# Autodesk Inventor assembly: パネル型スカラアーム
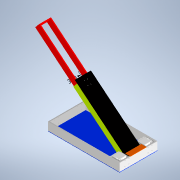
[picture p0: Inventor's stored thumbnail of the model, 180x180]
Saved by Autodesk Inventor 2022 (Build 260153000, 153)
## iProperties
Created: 2022-10-17
Part Number: パネル型スカラアーム
Document SubType Name: Assembly
Designer: tdn82
Mass: 1402.96 g
Surface Area: 5352.73 cm^2
Volume: 859.492 cm^3
Density: 1.63232 g/cm^3
Author: tdn82
## Documents named in this file (14)
- C:\Users\tdn82\OneDrive\ドキュメント\Inventor\卒業研究パネル型スカラアーム\GrabCAD\panel-type-scalar-arm\パネル型スカラアーム\パネル型スカラアーム.iam
- C:\Users\tdn82\OneDrive\ドキュメント\Inventor\卒業研究パネル型スカラアーム\GrabCAD\panel-type-scalar-arm\パネル型スカラアーム\縦長フラットバー.ipt
- C:\Users\tdn82\OneDrive\ドキュメント\Inventor\卒業研究パネル型スカラアーム\GrabCAD\panel-type-scalar-arm\パネル型スカラアーム\横長フラットバー.ipt
- C:\Users\tdn82\OneDrive\ドキュメント\Inventor\卒業研究パネル型スカラアーム\GrabCAD\panel-type-scalar-arm\パネル型スカラアーム\サーボモータB3M-SC-1170-AB3M1100_scale.ipt
- C:\Users\tdn82\OneDrive\ドキュメント\Inventor\卒業研究パネル型スカラアーム\GrabCAD\panel-type-scalar-arm\パネル型スカラアーム\後ろカバー.ipt
- C:\Users\tdn82\OneDrive\ドキュメント\Inventor\卒業研究パネル型スカラアーム\GrabCAD\panel-type-scalar-arm\パネル型スカラアーム\横長3rdフラットバー.ipt
- C:\Users\tdn82\OneDrive\ドキュメント\Inventor\卒業研究パネル型スカラアーム\GrabCAD\panel-type-scalar-arm\パネル型スカラアーム\縦長3rdフラットバー.ipt
- C:\Users\tdn82\OneDrive\ドキュメント\Inventor\卒業研究パネル型スカラアーム\GrabCAD\panel-type-scalar-arm\パネル型スカラアーム\１段目アーム.iam
- C:\Users\tdn82\OneDrive\ドキュメント\Inventor\卒業研究パネル型スカラアーム\GrabCAD\panel-type-scalar-arm\パネル型スカラアーム\横長2ndフラットバー.ipt
- C:\Users\tdn82\OneDrive\ドキュメント\Inventor\卒業研究パネル型スカラアーム\GrabCAD\panel-type-scalar-arm\パネル型スカラアーム\横長3rdフラットバー上.ipt
- C:\Users\tdn82\OneDrive\ドキュメント\Inventor\卒業研究パネル型スカラアーム\GrabCAD\panel-type-scalar-arm\パネル型スカラアーム\サーボモータ固定２軸目.ipt
- C:\Users\tdn82\OneDrive\ドキュメント\Inventor\卒業研究パネル型スカラアーム\GrabCAD\panel-type-scalar-arm\パネル型スカラアーム\前上下カバー.ipt
- C:\Users\tdn82\OneDrive\ドキュメント\Inventor\卒業研究パネル型スカラアーム\GrabCAD\panel-type-scalar-arm\パネル型スカラアーム\前カバー中盤.ipt
- C:\Users\tdn82\OneDrive\ドキュメント\Inventor\卒業研究パネル型スカラアーム\GrabCAD\panel-type-scalar-arm\パネル型スカラアーム\黒棒.ipt
## Components (18 placed, 13 different names)
1. 縦長フラットバー:1 — メイト:1, フラッシュ:1, フラッシュ:2, フラッシュ:3, メイト:2, メイト:3, メイト:4, メイト:12
2. 縦長フラットバー:2 — メイト:5, メイト:6, メイト:7, メイト:8, 挿入:1, 挿入:2, 挿入:3, 挿入:4, メイト:22, メイト:24, メイト:29, メイト:31
3. 横長フラットバー:1 — メイト:2, メイト:3, メイト:4, メイト:5, メイト:6, メイト:11, メイト:23
4. 横長フラットバー:3 — メイト:7, メイト:8, メイト:25
5. サーボモータB3M-SC-1170-AB3M1100_scale:2 — 挿入:7, 挿入:8, 挿入:9
6. 後ろカバー:1 — メイト:11, メイト:12
7. 横長3rdフラットバー:2 — メイト:18, メイト:19, 挿入:7
8. 縦長3rdフラットバー:1 — メイト:18, メイト:19, メイト:20, メイト:21
9. １段目アーム:1 [sub-assembly] — 挿入:1, 挿入:2, 挿入:12
10. １段目アーム:2 [sub-assembly] — 挿入:3, 挿入:4, 挿入:13
11. 横長2ndフラットバー:1 — フラッシュ:4, 挿入:13
12. 横長2ndフラットバー:2 — フラッシュ:4, メイト:26, メイト:27, メイト:28, 挿入:12
13. 横長3rdフラットバー上:1 — メイト:20, メイト:21
14. 前上下カバー:1 — メイト:22, メイト:23, メイト:30
15. 前上下カバー:2 — メイト:24, メイト:25
16. 前カバー中盤:1 — メイト:26, メイト:27, メイト:28, 挿入:10, 挿入:11
17. サーボモータ固定２軸目:1 — 挿入:8, 挿入:9, 挿入:10, 挿入:11
18. 黒棒:1 — メイト:29, メイト:30, メイト:31
## Relationships (39: Mate 24, Insert 11, Flush 4)
- メイト:1 [Mate]: 縦長フラットバー:1
- フラッシュ:1 [Flush]: 縦長フラットバー:1
- フラッシュ:2 [Flush]: 縦長フラットバー:1
- フラッシュ:3 [Flush]: 縦長フラットバー:1
- メイト:2 [Mate]: 縦長フラットバー:1 ↔ 横長フラットバー:1
- メイト:3 [Mate]: 縦長フラットバー:1 ↔ 横長フラットバー:1
- メイト:4 [Mate]: 縦長フラットバー:1 ↔ 横長フラットバー:1
- メイト:5 [Mate]: 縦長フラットバー:2 ↔ 横長フラットバー:1
- メイト:6 [Mate]: 縦長フラットバー:2 ↔ 横長フラットバー:1
- メイト:7 [Mate]: 縦長フラットバー:2 ↔ 横長フラットバー:3
- メイト:8 [Mate]: 縦長フラットバー:2 ↔ 横長フラットバー:3
- メイト:11 [Mate]: 横長フラットバー:1 ↔ 後ろカバー:1
- メイト:12 [Mate]: 縦長フラットバー:1 ↔ 後ろカバー:1
- メイト:18 [Mate]: 横長3rdフラットバー:2 ↔ 縦長3rdフラットバー:1
- メイト:19 [Mate]: 横長3rdフラットバー:2 ↔ 縦長3rdフラットバー:1
- 挿入:1 [Insert]: 縦長フラットバー:2 ↔ １段目アーム:1
- 挿入:2 [Insert]: 縦長フラットバー:2 ↔ １段目アーム:1
- 挿入:3 [Insert]: 縦長フラットバー:2 ↔ １段目アーム:2
- 挿入:4 [Insert]: 縦長フラットバー:2 ↔ １段目アーム:2
- フラッシュ:4 [Flush]: 横長2ndフラットバー:1 ↔ 横長2ndフラットバー:2
- 挿入:7 [Insert]: サーボモータB3M-SC-1170-AB3M1100_scale:2 ↔ 横長3rdフラットバー:2
- メイト:20 [Mate]: 縦長3rdフラットバー:1 ↔ 横長3rdフラットバー上:1
- メイト:21 [Mate]: 縦長3rdフラットバー:1 ↔ 横長3rdフラットバー上:1
- メイト:22 [Mate]: 縦長フラットバー:2 ↔ 前上下カバー:1
- メイト:23 [Mate]: 横長フラットバー:1 ↔ 前上下カバー:1
- メイト:24 [Mate]: 縦長フラットバー:2 ↔ 前上下カバー:2
- メイト:25 [Mate]: 横長フラットバー:3 ↔ 前上下カバー:2
- 挿入:8 [Insert]: サーボモータB3M-SC-1170-AB3M1100_scale:2 ↔ サーボモータ固定２軸目:1
- 挿入:9 [Insert]: サーボモータB3M-SC-1170-AB3M1100_scale:2 ↔ サーボモータ固定２軸目:1
- メイト:26 [Mate]: 横長2ndフラットバー:2 ↔ 前カバー中盤:1
- メイト:27 [Mate] (0.5 mm): 横長2ndフラットバー:2 ↔ 前カバー中盤:1
- メイト:28 [Mate] (11 mm): 横長2ndフラットバー:2 ↔ 前カバー中盤:1
- 挿入:10 [Insert]: 前カバー中盤:1 ↔ サーボモータ固定２軸目:1
- 挿入:11 [Insert]: 前カバー中盤:1 ↔ サーボモータ固定２軸目:1
- メイト:29 [Mate]: 縦長フラットバー:2 ↔ 黒棒:1
- メイト:30 [Mate]: 前上下カバー:1 ↔ 黒棒:1
- メイト:31 [Mate]: 縦長フラットバー:2 ↔ 黒棒:1
- 挿入:12 [Insert]: １段目アーム:1 ↔ 横長2ndフラットバー:2
- 挿入:13 [Insert]: １段目アーム:2 ↔ 横長2ndフラットバー:1
